# Autodesk Inventor assembly: ASY HPR 350 Auger
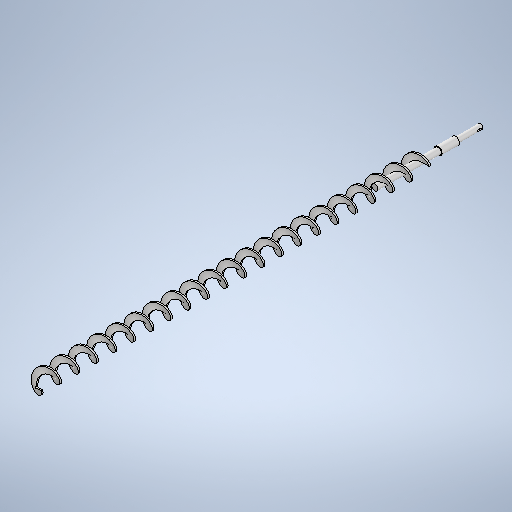
[picture p0: Inventor's stored thumbnail of the model, 512x512]
Saved by Autodesk Inventor 2025.1 (Build 291241020, 241B)
## iProperties
Created: 2025-04-01
Part Number: ASY HPR 350 Auger
Document SubType Name: Assembly
Designer: user
Author: user
## Documents named in this file (3)
- C:\Users\user\YandexDisk-badmisterfox\home pc\Inventor\NDM-VOS_powder_hopper\ASY HPR 350 Auger.iam
- C:\Users\user\YandexDisk-badmisterfox\home pc\Inventor\NDM-VOS_powder_hopper\NVPH-401 auger.ipt
- C:\Users\user\YandexDisk-badmisterfox\home pc\Inventor\NDM-VOS_powder_hopper\NVPH-502 augur shaft.ipt
## Components (2 placed, 2 different names)
1. NVPH-401 auger:1
2. NVPH-502 augur shaft:1
## Relationships (1: WeldJoint 1)
- [WeldJoint] (80 mm): NVPH-401 auger:1 ↔ NVPH-502 augur shaft:1
